# Autodesk Inventor assembly: sestava_auto
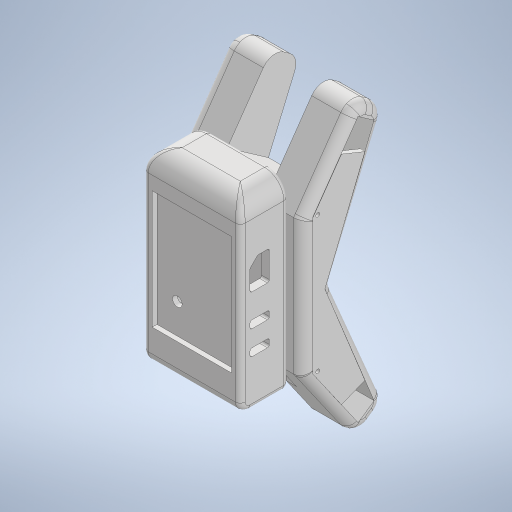
[picture p0: Inventor's stored thumbnail of the model, 512x512]
Saved by Autodesk Inventor 2024 (Build 280153000, 153)
## iProperties
Created: 2024-03-06
Part Number: sestava_auto
Document SubType Name: Assembly
Designer: Game
Author: Game
## Documents named in this file (4)
- D:\Users\Desktop\auto_model\sestava_auto.iam
- D:\Users\Desktop\auto_model\karoserie.ipt
- D:\Users\Desktop\auto_model\podvozek.ipt
- D:\Users\Desktop\auto_model\zaver.ipt
## Components (4 placed, 3 different names)
1. karoserie:1 — Tuhé:1
2. podvozek:1 — Tuhé:1, Tuhé:2, Tuhé:3
3. zaver:1 — Tuhé:3
4. zaver:2 — Tuhé:2
## Relationships (3: WeldJoint 3)
- Tuhé:1 [WeldJoint]: karoserie:1 ↔ podvozek:1
- Tuhé:2 [WeldJoint]: podvozek:1 ↔ zaver:2
- Tuhé:3 [WeldJoint]: podvozek:1 ↔ zaver:1
